# Autodesk Inventor assembly: EDMPumpRegionAssembly
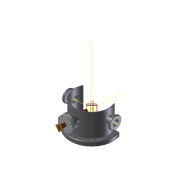
[picture p0: Inventor's stored thumbnail of the model, 180x180]
Saved by Autodesk Inventor 2015 (Build 190159000, 159)
## iProperties
Created: 2014-03-24
Part Number: EDMPumpRegionAssembly
Document SubType Name: Assembly
Designer: jad211
Author: jad211
## Documents named in this file (7)
- C:\CADFiles\EDM Machine\EDM New Pumping Region\EDMPumpRegionAssembly.iam
- C:\CADFiles\EDM Machine\EDM Middle Shield\EDM Middle shield.ipt
- C:\CADFiles\EDM Machine\EDM Inner Shield\Inner Shield.iam
- C:\CADFiles\EDM Machine\EDM Beamline\Chamber parts\hudson chamber actual size.ipt
- C:\CADFiles\EDM Machine\EDM New Pumping Region\StraightPumpRegion.iam
- C:\CADFiles\EDM Machine\EDM New Pumping Region\rfCoil.ipt
- C:\CADFiles\EDM Machine\EDM New Pumping Region\rfCoilSmaller.ipt
## Components (8 placed, 6 different names)
1. EDM Middle shield:1 — Mate:8, Flush:11
2. Inner Shield:1 [sub-assembly] — Flush:14, Mate:10, Flush:13, Flush:19
3. hudson chamber actual size:1 — Mate:12, Flush:15, Angle:1, Mate:13, Mate:14, Mate:15, Mate:18, Mate:19, Mate:20
4. StraightPumpRegion:1 [sub-assembly] — Angle:2, Flush:20, Mate:14
5. rfCoil:1 — Mate:29, Mate:30, Mate:31, Mate:32
6. rfCoil:2 — Mate:26, Mate:27, Mate:28, Mate:29, Mate:30, Mate:31, Mate:32
7. rfCoilSmaller:1 — Mate:16, Mate:17, Mate:21, Mate:22, Mate:23, Mate:24, Mate:25, Mate:33, Mate:34, Mate:35, Mate:36
8. rfCoilSmaller:2 — Mate:22, Mate:23, Mate:24, Mate:25, Mate:33, Mate:34, Mate:35, Mate:36
## Relationships (39: Mate 27, Flush 8, Angle 4)
- Flush:8 (3 mm)
- Mate:8: EDM Middle shield:1
- Flush:11 (158.75 mm): EDM Middle shield:1
- Flush:14 (64.29 mm): Inner Shield:1
- Mate:10: Inner Shield:1
- Flush:13: Inner Shield:1
- Mate:12: hudson chamber actual size:1
- Flush:15: hudson chamber actual size:1
- Flush:16 (-304.8 mm)
- Angle:1 (0 deg): hudson chamber actual size:1
- Mate:13: hudson chamber actual size:1
- Flush:19 (90 mm): Inner Shield:1
- Angle:2 (0 deg): StraightPumpRegion:1
- Flush:20 (-30 mm): StraightPumpRegion:1
- Mate:14: hudson chamber actual size:1 ↔ StraightPumpRegion:1
- Mate:15: hudson chamber actual size:1
- Angle:3 (45 deg)
- Mate:16 (5 mm): rfCoilSmaller:1
- Mate:17 (5 mm): rfCoilSmaller:1
- Mate:18: hudson chamber actual size:1
- Angle:4 (90 deg)
- Mate:19: hudson chamber actual size:1
- Mate:20: hudson chamber actual size:1
- Mate:21 (22.5 mm): rfCoilSmaller:1
- Mate:22 (10 mm): rfCoilSmaller:1 ↔ rfCoilSmaller:2
- Mate:23 (10 mm): rfCoilSmaller:1 ↔ rfCoilSmaller:2
- Mate:24 (10 mm): rfCoilSmaller:1 ↔ rfCoilSmaller:2
- Mate:25 (10 mm): rfCoilSmaller:1 ↔ rfCoilSmaller:2
- Mate:26 (5 mm): rfCoil:2
- Mate:27 (5 mm): rfCoil:2
- Mate:28 (25 mm): rfCoil:2
- Mate:29 (10 mm): rfCoil:1 ↔ rfCoil:2
- Mate:30 (10 mm): rfCoil:1 ↔ rfCoil:2
- Mate:31 (10 mm): rfCoil:1 ↔ rfCoil:2
- Mate:32 (10 mm): rfCoil:1 ↔ rfCoil:2
- Mate:33 (10 mm): rfCoilSmaller:1 ↔ rfCoilSmaller:2
- Mate:34 (10 mm): rfCoilSmaller:1 ↔ rfCoilSmaller:2
- Mate:35 (10 mm): rfCoilSmaller:1 ↔ rfCoilSmaller:2
- Mate:36 (10 mm): rfCoilSmaller:1 ↔ rfCoilSmaller:2
